# Autodesk Inventor assembly: SoldeerstationAssambly
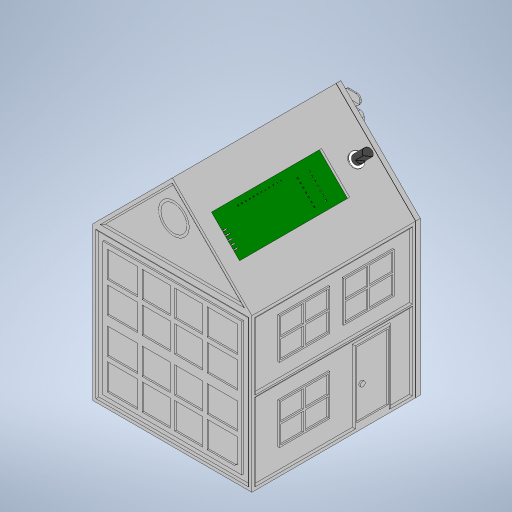
[picture p0: Inventor's stored thumbnail of the model, 512x512]
Saved by Autodesk Inventor 2023 (Build 270158000, 158)
## iProperties
Created: 2023-05-29
Part Number: SoldeerstationAssambly
Document SubType Name: Assembly
Designer: jaspe
Author: jaspe
## Documents named in this file (8)
- C:\Users\jaspe\OneDrive - PXL\Documenten\Electonica-ICT-1e jaar\Project ontwerpen\Ontwerpen\Soldeerstation2\SoldeerstationAssambly.iam
- C:\Users\jaspe\OneDrive - PXL\Documenten\Electonica-ICT-1e jaar\Project ontwerpen\Ontwerpen\Soldeerstation2\HouseSolderingStation.ipt
- C:\Users\jaspe\OneDrive - PXL\Documenten\Electonica-ICT-1e jaar\Project ontwerpen\Ontwerpen\Soldeerstation2\DekselCase.ipt
- C:\Users\jaspe\OneDrive - PXL\Documenten\Electonica-ICT-1e jaar\Project ontwerpen\Ontwerpen\Soldeerstation2\Soldeerstation.iam
- C:\Users\jaspe\OneDrive - PXL\Documenten\Electonica-ICT-1e jaar\Project ontwerpen\Ontwerpen\Soldeerstation2\TraFo.ipt
- C:\Users\jaspe\OneDrive - PXL\Documenten\Electonica-ICT-1e jaar\Project ontwerpen\Ontwerpen\Soldeerstation2\PCB2.iam
- C:\Users\jaspe\OneDrive - PXL\Documenten\Electonica-ICT-1e jaar\Project ontwerpen\Ontwerpen\Soldeerstation2\power connector.ipt
- C:\Users\jaspe\OneDrive - PXL\Documenten\Electonica-ICT-1e jaar\Project ontwerpen\Ontwerpen\Neutrik 4Pin Panel Mount Female.ipt
## Components (7 placed, 7 different names)
1. HouseSolderingStation:1 — Mate:1, Mate:2, Mate:3, Mate:4, Mate:5, Mate:6
2. DekselCase:1 — Mate:1, Mate:6, Insert:1
3. Soldeerstation:1 [sub-assembly] — Mate:2
4. TraFo:1 — Mate:3
5. PCB2:1 [sub-assembly]
6. power connector:1 — Mate:4, Mate:5
7. Neutrik 4Pin Panel Mount Female:1 — Insert:1
## Relationships (7: Mate 6, Insert 1)
- Mate:1: HouseSolderingStation:1 ↔ DekselCase:1
- Mate:2: HouseSolderingStation:1 ↔ Soldeerstation:1
- Mate:3: HouseSolderingStation:1 ↔ TraFo:1
- Mate:4: HouseSolderingStation:1 ↔ power connector:1
- Mate:5: HouseSolderingStation:1 ↔ power connector:1
- Mate:6: HouseSolderingStation:1 ↔ DekselCase:1
- Insert:1: DekselCase:1 ↔ Neutrik 4Pin Panel Mount Female:1
